# Autodesk Inventor assembly: Fridge-Full
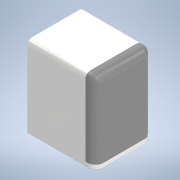
[picture p0: Inventor's stored thumbnail of the model, 180x180]
Saved by Autodesk Inventor 2020 (Build 240168000, 168)
## iProperties
Created: 2020-02-07
Part Number: Fridge-Full
Document SubType Name: Assembly
Designer: Simon
Author: Simon
## Documents named in this file (3)
- D:\Simon\vroomvroom\Fridge\Fridge-Full.iam
- D:\Simon\vroomvroom\Fridge\Fridge-Body.ipt
- D:\Simon\vroomvroom\Fridge\Fridge-Door.ipt
## Components (2 placed, 2 different names)
1. Fridge-Body:1 — Rotational:1
2. Fridge-Door:1 — Rotational:1
## Relationships (1: RevoluteJoint 1)
- Rotational:1 [RevoluteJoint]: Fridge-Body:1 ↔ Fridge-Door:1
